# Autodesk Inventor assembly: SAR330 + regular couplers right offset
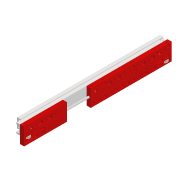
[picture p0: Inventor's stored thumbnail of the model, 180x180]
Saved by Autodesk Inventor 2020 (Build 240168000, 168)
## iProperties
Created: 2019-12-12
Part Number: SAR330 + regular couplers right offset
Document SubType Name: Assembly
Designer: ball
Author: ball
## Documents named in this file (5)
- C:\FTC\FTC8863CAD\2019 Robot\Delivery\Lift Right\SAR330 + regular couplers right offset.iam
- C:\FTC\FTC8863CAD\2019 Robot\Delivery\Lift Right\Coupler lift long right + pulleys.iam
- C:\FTC\FTC8863CAD\Misumi\SAR330\SAR330 440 offset.iam
- C:\FTC\FTC8863CAD\2019 Robot\Delivery\Lift Right\Coupler lift short right + pulleys.iam
- C:\FTC\FTC8863CAD\Actobotics\634 parts\634266.ipt
## Components (4 placed, 4 different names)
1. SAR330 440 offset:1 [sub-assembly] — Mate:1, Mate:2, Mate:3, Mate:4, Mate:5, Flush:1
2. Coupler lift long right + pulleys:1 [sub-assembly] — Mate:1, Mate:2, Mate:3, Mate:6
3. Coupler lift short right + pulleys:1 [sub-assembly] — Mate:4, Mate:5, Flush:1, Mate:7
4. 634266:1 — Mate:6, Mate:7
## Relationships (8: Mate 7, Flush 1)
- Mate:1: SAR330 440 offset:1 ↔ Coupler lift long right + pulleys:1
- Mate:2: SAR330 440 offset:1 ↔ Coupler lift long right + pulleys:1
- Mate:3: SAR330 440 offset:1 ↔ Coupler lift long right + pulleys:1
- Mate:4: SAR330 440 offset:1 ↔ Coupler lift short right + pulleys:1
- Mate:5: SAR330 440 offset:1 ↔ Coupler lift short right + pulleys:1
- Flush:1: SAR330 440 offset:1 ↔ Coupler lift short right + pulleys:1
- Mate:6: Coupler lift long right + pulleys:1 ↔ 634266:1
- Mate:7: Coupler lift short right + pulleys:1 ↔ 634266:1
